# Autodesk Inventor assembly: sensor
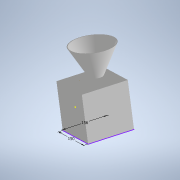
[picture p0: Inventor's stored thumbnail of the model, 180x180]
Saved by Autodesk Inventor 2020 (Build 240168000, 168)
## iProperties
Created: 2020-12-15
Part Number: sensor
Document SubType Name: Assembly
Designer: moham
Author: moham
## Documents named in this file (10)
- D:\Projects\MCT 131\The project\sensor.iam
- D:\Projects\MCT 131\The project\box side.ipt
- D:\Projects\MCT 131\The project\cone.ipt
- D:\Projects\MCT 131\The project\Part10.ipt
- D:\Projects\MCT 131\The project\box top.ipt
- D:\Projects\MCT 131\The project\tube.ipt
- D:\Projects\MCT 131\The project\Rotator.ipt
- D:\Projects\MCT 131\The project\Holder.ipt
- D:\Projects\MCT 131\The project\box bottom.ipt
- D:\Projects\MCT 131\The project\holder2.ipt
## Components (13 placed, 9 different names)
1. Part10:1
2. box top:1 — Mate:1, Mate:2, Flush:8, Flush:9, Mate:12, Mate:13
3. cone:1 — Mate:1, Mate:2, Mate:14
4. box side:1 — Mate:10, Mate:11, Flush:5, Flush:6, Flush:7, Flush:9, Flush:11
5. box side:2 — Mate:9, Flush:3, Flush:4, Mate:10, Flush:6, Flush:7, Flush:8, Mate:12, Flush:10
6. box side:3 — Mate:8, Flush:1, Flush:2, Mate:9, Flush:3, Flush:4, Mate:21
7. box side:4 — Mate:8, Flush:1, Flush:2, Mate:11, Flush:5, Flush:12
8. tube:1 — Mate:13, Mate:14, Rigid:2
9. Rotator:1 — Rotational:2
10. Holder:1 — Rotational:2, Rigid:2
11. box bottom:1 — Mate:21, Flush:10, Flush:11, Flush:12, Mate:23, Mate:26
12. holder2:1 — Mate:23
13. holder2:2 — Mate:26
## Relationships (26: Mate 12, Flush 12, RevoluteJoint 1, WeldJoint 1)
- Mate:1: box top:1 ↔ cone:1
- Mate:2: box top:1 ↔ cone:1
- Mate:8: box side:3 ↔ box side:4
- Flush:1: box side:3 ↔ box side:4
- Flush:2: box side:3 ↔ box side:4
- Mate:9: box side:2 ↔ box side:3
- Flush:3: box side:2 ↔ box side:3
- Flush:4: box side:2 ↔ box side:3
- Mate:10: box side:1 ↔ box side:2
- Mate:11: box side:1 ↔ box side:4
- Flush:5: box side:1 ↔ box side:4
- Flush:6: box side:1 ↔ box side:2
- Flush:7: box side:1 ↔ box side:2
- Flush:8: box top:1 ↔ box side:2
- Flush:9: box top:1 ↔ box side:1
- Mate:12: box top:1 ↔ box side:2
- Mate:13: box top:1 ↔ tube:1
- Mate:14: cone:1 ↔ tube:1
- Mate:21: box side:3 ↔ box bottom:1
- Flush:10: box side:2 ↔ box bottom:1
- Flush:11: box side:1 ↔ box bottom:1
- Flush:12: box side:4 ↔ box bottom:1
- Mate:23: box bottom:1 ↔ holder2:1
- Mate:26: box bottom:1 ↔ holder2:2
- Rotational:2 [RevoluteJoint] (-20 mm): Rotator:1 ↔ Holder:1
- Rigid:2 [WeldJoint] (45 mm): tube:1 ↔ Holder:1
